# Autodesk Inventor assembly: CSL_AQS_V1_spin3 1
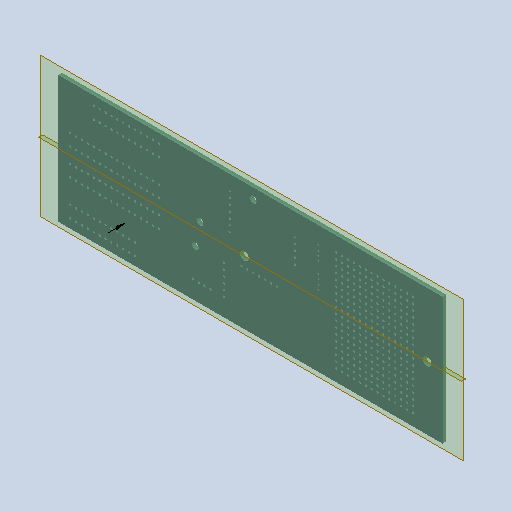
[picture p0: Inventor's stored thumbnail of the model, 512x512]
Saved by Autodesk Inventor 2025.3 (Build 293356000, 356)
## iProperties
Company: Kicad
Created: 2024-06-25
Part Number: CSL_AQS_V1_spin3 1
Description: KiCad electronic assembly
Document SubType Name: Assembly
Designer: vncnt
Authority: Unknown
Sending System: KiCad to STEP converter
Preprocessor: Open CASCADE STEP processor 7.8
Title: CSL_AQS_V1_spin3.step
Author: Pcbnew
## Documents named in this file (2)
- C:\Users\vncnt\OneDrive\Documents\Inventor\ASRC\Air Quality Sensor\Air Quality Board Mount\CSL AQS V1 spin3.iam
- C:\Users\vncnt\OneDrive\Documents\Inventor\ASRC\Air Quality Sensor\Air Quality Board Mount\CSL AQS V1 PCB.ipt
## Components (1 placed, 1 different names)
1. 13 — Flush:1, Flush:2
## Relationships (2: Flush 2)
- Flush:1 (-27.305 mm): 13
- Flush:2 (-0.8 mm): 13
